# Autodesk Inventor assembly: PCB enclosure
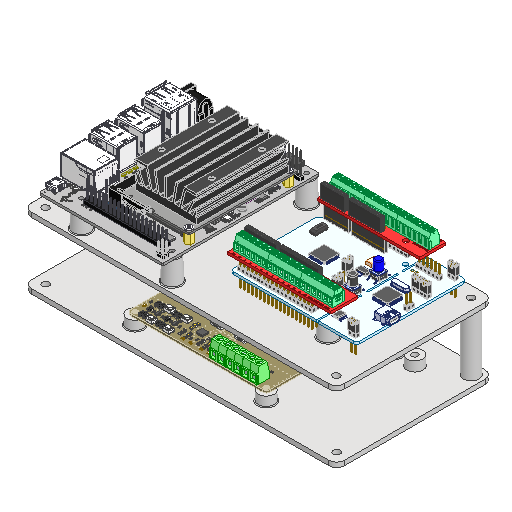
[picture p0: Inventor's stored thumbnail of the model, 512x512]
Saved by Autodesk Inventor 2026 (Build 300175050, 175E)
## iProperties
Created: 2025-10-28
Part Number: PCB enclosure
Document SubType Name: Assembly
Designer: Kartik
Mass: 238.616 g
Surface Area: 2576.37 cm^2
Volume: 238.616 cm^3
Density: 1 g/cm^3
Author: Kartik
## Documents named in this file (9)
- D:\Kartik\Projects\AMR\CAD\Sub-assembly\PCB enclosure.iam
- D:\Kartik\Projects\AMR\CAD\MDD20A CAD\MDD20A\MDD20A\MDD20A.ipt
- D:\Kartik\Projects\AMR\CAD\Boughtouts\NUCLEO-F401RE--3DModel-STEP-56544\NUCLEO-F401RE--3DModel-STEP-56544\NUCLEO-F401RE--3DModel-STEP-56544.ipt
- D:\Kartik\Projects\AMR\CAD\Boughtouts\NUCLEO-F401RE--3DModel-STEP-56544\Arduino UNO R3 screw Shield v2 Left\Arduino UNO R3 screw Shield v2 Left.ipt
- D:\Kartik\Projects\AMR\CAD\Boughtouts\NUCLEO-F401RE--3DModel-STEP-56544\Arduino UNO R3 screw Shield v2 Right\Arduino UNO R3 screw Shield v2 Right.ipt
- D:\Kartik\Projects\AMR\CAD\Boughtouts\nvidia-jetson-nano-4gb\Jetson nano 4GB\Jetson nano 4GB\Jetson nano 4GB.ipt
- D:\Kartik\Projects\AMR\CAD\Parts\Base_MDD20A.ipt
- D:\Kartik\Projects\AMR\CAD\Parts\Base_ST_nano.ipt
- D:\Kartik\Projects\AMR\CAD\Parts\Spacer.ipt
## Components (8 placed, 8 different names)
1. MDD20A:1 — Mate:1, Flush:8, Mate:7, Mate:8, Mate:9, Angle:2
2. NUCLEO-F401RE--3DModel-STEP-56544:1 — Mate:1, Mate:2, Flush:3, Flush:4, Mate:3, Flush:5, Flush:6, Flush:9, Flush:8, Mate:6, Mate:17, Mate:18
3. Arduino UNO R3 screw Shield v2 Left:1 — Mate:2, Flush:3, Flush:4
4. Arduino UNO R3 screw Shield v2 Right:1 — Mate:3, Flush:5, Flush:6
5. Jetson nano 4GB:1 — Flush:9, Angle:1, Mate:11, Mate:15, Mate:16
6. Base_MDD20A:1 — Mate:7, Mate:8, Mate:9, Angle:2, Flush:10, Mate:19, Mate:20
7. Base_ST_nano:1 — Mate:11, Flush:10, Mate:15, Mate:16, Mate:17, Mate:18
8. Spacer:1 — Mate:19, Mate:20
## Relationships (23: Mate 14, Flush 7, Angle 2)
- Mate:1 (50 mm): MDD20A:1 ↔ NUCLEO-F401RE--3DModel-STEP-56544:1
- Mate:2: NUCLEO-F401RE--3DModel-STEP-56544:1 ↔ Arduino UNO R3 screw Shield v2 Left:1
- Flush:3: NUCLEO-F401RE--3DModel-STEP-56544:1 ↔ Arduino UNO R3 screw Shield v2 Left:1
- Flush:4: NUCLEO-F401RE--3DModel-STEP-56544:1 ↔ Arduino UNO R3 screw Shield v2 Left:1
- Mate:3: NUCLEO-F401RE--3DModel-STEP-56544:1 ↔ Arduino UNO R3 screw Shield v2 Right:1
- Flush:5: NUCLEO-F401RE--3DModel-STEP-56544:1 ↔ Arduino UNO R3 screw Shield v2 Right:1
- Flush:6: NUCLEO-F401RE--3DModel-STEP-56544:1 ↔ Arduino UNO R3 screw Shield v2 Right:1
- Flush:9: NUCLEO-F401RE--3DModel-STEP-56544:1 ↔ Jetson nano 4GB:1
- Flush:8: MDD20A:1 ↔ NUCLEO-F401RE--3DModel-STEP-56544:1
- Angle:1 (0 deg): Jetson nano 4GB:1
- Mate:6: NUCLEO-F401RE--3DModel-STEP-56544:1
- Mate:7: MDD20A:1 ↔ Base_MDD20A:1
- Mate:8 (-2.5 mm): MDD20A:1 ↔ Base_MDD20A:1
- Mate:9 (-2.5 mm): MDD20A:1 ↔ Base_MDD20A:1
- Angle:2 (0 deg): MDD20A:1 ↔ Base_MDD20A:1
- Mate:11: Jetson nano 4GB:1 ↔ Base_ST_nano:1
- Flush:10: Base_MDD20A:1 ↔ Base_ST_nano:1
- Mate:15: Jetson nano 4GB:1 ↔ Base_ST_nano:1
- Mate:16: Jetson nano 4GB:1 ↔ Base_ST_nano:1
- Mate:17: NUCLEO-F401RE--3DModel-STEP-56544:1 ↔ Base_ST_nano:1
- Mate:18: NUCLEO-F401RE--3DModel-STEP-56544:1 ↔ Base_ST_nano:1
- Mate:19: Base_MDD20A:1 ↔ Spacer:1
- Mate:20: Base_MDD20A:1 ↔ Spacer:1
